# Autodesk Inventor assembly: PWTR-0145
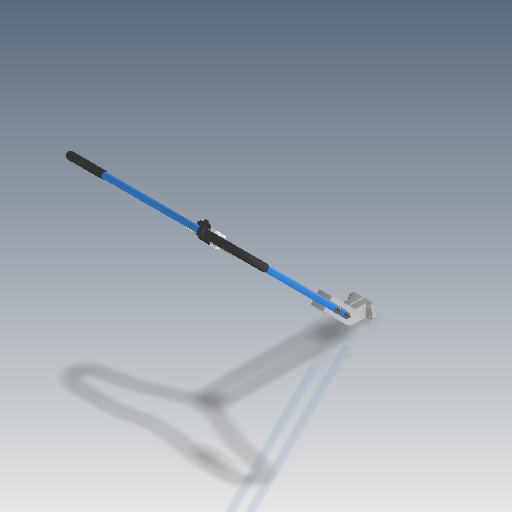
[picture p0: Inventor's stored thumbnail of the model, 512x512]
Saved by Autodesk Inventor 2021.1 (Build 251245000, 245)
## iProperties
Created: 2020-08-28
Part Number: PWTR-0145
Document SubType Name: Assembly
Designer: alid
Description: Handle Assembly
Author: alid
Revision Number: A
## Documents named in this file (9)
- C:\Vault Workspace\Design Data\Projects\PRJ0095\PWTR-CTO\PWTR-0145.iam
- C:\Vault Workspace\Design Data\Projects\PRJ0095\PWTR-CTO\PWTR-Supplier\PWTR-Controls\PWTR-0103.iam
- C:\Vault Workspace\Design Data\Projects\PRJ0095\PWTR-CTO\PWTR-0113.ipt
- C:\Vault Workspace\Design Data\Projects\PRJ0095\PWTR-CTO\PWTR-0117.ipt
- C:\Vault Workspace\Design Data\Projects\PRJ0095\PWTR-CTO\PWTR-0144.ipt
- C:\Vault Workspace\Design Data\Projects\PRJ0095\PWTR-CTO\PWTR-Supplier\PWTR-Controls\PWTR-0146.ipt
- C:\Vault Workspace\Design Data\Projects\PRJ0095\PWTR-CTO\PWTR-0147.iam
- C:\Vault Workspace\Design Data\Projects\PRJ0095\PWTR-CTO\PWTR-0151.ipt
- C:\Vault Workspace\Design Data\Projects\PRJ0095\PWTR-CTO\PWTR-0152.ipt
## Components (10 placed, 8 different names)
1. HandleConn — Rigid:7
2. Arm — Rigid:6, Rigid:7, Rigid:8, Rigid:9, Mate:1, Mate:2, Rigid:10
3. PWTR-0103:1 [sub-assembly] — Rigid:6
4. PWTR-0113:1 — Insert:6, Insert:8
5. PWTR-0117:1 — Insert:6, Insert:9, Angle:1
6. PWTR-0147:2 [sub-assembly] — Rigid:8
7. PWTR-0147:1 [sub-assembly] — Rigid:9
8. PWTR-0151:1 — Mate:1, Mate:2, Mate:3, Insert:8
9. PWTR-0147:3 [sub-assembly] — Rigid:10, Mate:3
10. PWTR-0152:1 — Insert:9, Angle:1
## Relationships (12: WeldJoint 5, Insert 3, Mate 3, Angle 1)
- Insert:6: PWTR-0113:1 ↔ PWTR-0117:1
- Rigid:6 [WeldJoint] (-5 mm): Arm ↔ PWTR-0103:1
- Rigid:7 [WeldJoint]: HandleConn ↔ Arm
- Rigid:8 [WeldJoint]: Arm ↔ PWTR-0147:2
- Rigid:9 [WeldJoint]: Arm ↔ PWTR-0147:1
- Mate:1: Arm ↔ PWTR-0151:1
- Mate:2: Arm ↔ PWTR-0151:1
- Rigid:10 [WeldJoint]: Arm ↔ PWTR-0147:3
- Mate:3: PWTR-0151:1 ↔ PWTR-0147:3
- Insert:8: PWTR-0113:1 ↔ PWTR-0151:1
- Insert:9: PWTR-0117:1 ↔ PWTR-0152:1
- Angle:1 (0 deg): PWTR-0117:1 ↔ PWTR-0152:1
